# Autodesk Inventor assembly: bottom idler housing
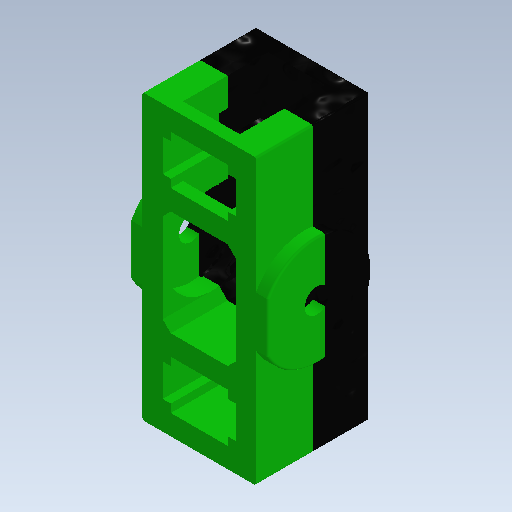
[picture p0: Inventor's stored thumbnail of the model, 512x512]
Saved by Autodesk Inventor 2020.4 (Build 244396000, 396)
## iProperties
Created: 2021-03-29
Part Number: bottom idler housing
Document SubType Name: Assembly
Designer: AOB
Mass: 32.4285 g
Surface Area: 168.027 cm^2
Volume: 30.5929 cm^3
Density: 1.06 g/cm^3
Author: AOB
## Documents named in this file (3)
- C:\Users\marti\Documents\Inventor\ProjectBoron\Boron Ultima\bottom idler housing.iam
- C:\Users\marti\Documents\Inventor\ProjectBoron\Boron Ultima\bottom idler housing-A.ipt
- C:\Users\marti\Documents\Inventor\ProjectBoron\Boron Ultima\bottom idler housing-B.ipt
## Components (2 placed, 2 different names)
1. bottom idler housing-A:1 — Flush:1, Flush:2, Rigid:1
2. bottom idler housing-B:1 — Flush:1, Flush:2, Rigid:1
## Relationships (3: Flush 2, WeldJoint 1)
- Flush:1: bottom idler housing-A:1 ↔ bottom idler housing-B:1
- Flush:2: bottom idler housing-A:1 ↔ bottom idler housing-B:1
- Rigid:1 [WeldJoint]: bottom idler housing-A:1 ↔ bottom idler housing-B:1
